# Autodesk Inventor assembly: Robot
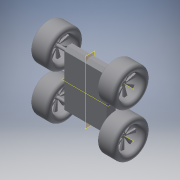
[picture p0: Inventor's stored thumbnail of the model, 180x180]
Saved by Autodesk Inventor 2018 (Build 220112000, 112)
## iProperties
Created: 2018-04-07
Part Number: Robot
Material: Générique
Document SubType Name: Assembly
Designer: Dimitri
Author: Dimitri
## Documents named in this file (10)
- C:\Users\Dimitri\Documents\Dimitri\Cours\Peip 2\Projet\Cao\Robot.iam
- C:\Users\Dimitri\Documents\Dimitri\Cours\Peip 2\Projet\Cao\Chassis.ipt
- C:\Users\Dimitri\Documents\Dimitri\Cours\Peip 2\Projet\Cao\Moteur roue.ipt
- C:\Users\Dimitri\Documents\Dimitri\Cours\Peip 2\Projet\Cao\Roue.ipt
- C:\Users\Dimitri\Documents\Dimitri\Cours\Peip 2\Projet\Cao\Moteur roue_MIR.ipt
- C:\Users\Dimitri\Documents\Dimitri\Cours\Peip 2\Projet\Cao\Roue_MIR.ipt
- C:\Users\Dimitri\Documents\Dimitri\Cours\Peip 2\Projet\Cao\Moteur roue_MIR1.ipt
- C:\Users\Dimitri\Documents\Dimitri\Cours\Peip 2\Projet\Cao\Roue_MIR1.ipt
- C:\Users\Dimitri\Documents\Dimitri\Cours\Peip 2\Projet\Cao\Moteur roue_MIR_MIR.ipt
- C:\Users\Dimitri\Documents\Dimitri\Cours\Peip 2\Projet\Cao\Roue_MIR_MIR.ipt
## Components (9 placed, 9 different names)
1. Chassis:1 — Placage:1, Tangente:1, Affleurement:3
2. Moteur roue:1 — Placage:1, Tangente:1, Affleurement:1, Placage:2
3. Roue:1 — Affleurement:1, Placage:2
4. Moteur roue_MIR:1 — Placage:3, Affleurement:2
5. Roue_MIR:1 — Placage:3, Affleurement:2
6. Moteur roue_MIR1:1 — Placage:4, Affleurement:4
7. Roue_MIR1:1 — Placage:4, Affleurement:4
8. Moteur roue_MIR_MIR:1 — Affleurement:5, Placage:5
9. Roue_MIR_MIR:1 — Affleurement:5, Placage:5
## Relationships (11: Mate 5, Flush 5, Tangent 1)
- Placage:1 [Mate]: Chassis:1 ↔ Moteur roue:1
- Tangente:1: Chassis:1 ↔ Moteur roue:1
- Affleurement:1 [Flush]: Moteur roue:1 ↔ Roue:1
- Placage:2 [Mate]: Moteur roue:1 ↔ Roue:1
- Placage:3 [Mate]: Moteur roue_MIR:1 ↔ Roue_MIR:1
- Affleurement:2 [Flush]: Moteur roue_MIR:1 ↔ Roue_MIR:1
- Affleurement:3 [Flush] (-95 mm): Chassis:1
- Placage:4 [Mate]: Moteur roue_MIR1:1 ↔ Roue_MIR1:1
- Affleurement:4 [Flush]: Moteur roue_MIR1:1 ↔ Roue_MIR1:1
- Affleurement:5 [Flush]: Moteur roue_MIR_MIR:1 ↔ Roue_MIR_MIR:1
- Placage:5 [Mate]: Moteur roue_MIR_MIR:1 ↔ Roue_MIR_MIR:1
